# Autodesk Inventor assembly: testRoboRescue_Chassis_Frame
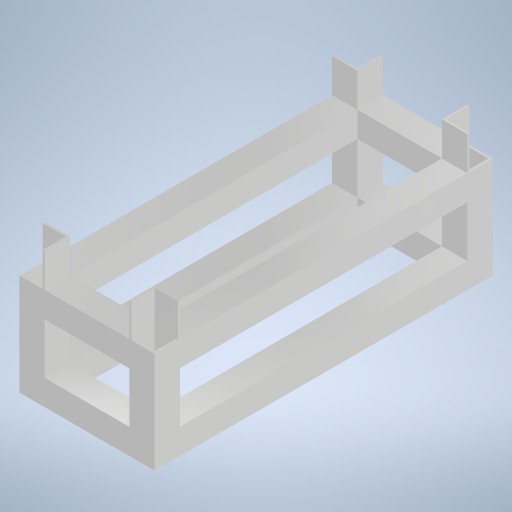
[picture p0: Inventor's stored thumbnail of the model, 512x512]
Saved by Autodesk Inventor 2023 (Build 270158000, 158)
## iProperties
Created: 2022-03-14
Part Number: testRoboRescue_Chassis_Frame
Document SubType Name: Assembly
Designer: Nebil Oumer
Mass: 3473.24 g
Surface Area: 8222.56 cm^2
Volume: 1286.38 cm^3
Author: Nebil Oumer
## Documents named in this file (5)
- C:\Users\seene\Desktop\Stony Brook\SBRT\RoboRescue\Chassis\Frame\testRoboRescue_Chassis_Frame.iam
- RoboRescue_Chassis_Frame.iam
- C:\Users\seene\Desktop\Stony Brook\SBRT\RoboRescue\Chassis\Frame\testRoboRescue_Chassis_Frame_heightBar.ipt
- C:\Users\seene\Desktop\Stony Brook\SBRT\RoboRescue\Chassis\Frame\testRoboRescue_Chassis_Frame_widthBar.ipt
- C:\Users\seene\Desktop\Stony Brook\SBRT\RoboRescue\Chassis\Frame\testRoboRescue_Chassis_Frame_lengthBar.ipt
## Components (12 placed, 3 different names)
1. testRoboRescue_Chassis_Frame_heightBar:1 — Mate:3, Flush:5, Flush:6, Flush:9, Flush:15, Mate:10, Flush:16, Mate:11, Mate:13, Mate:15, Flush:24
2. testRoboRescue_Chassis_Frame_heightBar:2 — Flush:1, Mate:1, Flush:2, Flush:3, Flush:4, Mate:2, Flush:21, Mate:14, Flush:22, Flush:23
3. testRoboRescue_Chassis_Frame_heightBar:3 — Mate:4, Flush:7, Flush:12, Mate:9, Flush:19
4. testRoboRescue_Chassis_Frame_heightBar:4 — Mate:5, Mate:6, Mate:7, Flush:11, Flush:13, Mate:8, Flush:14, Mate:12, Flush:20
5. testRoboRescue_Chassis_Frame_widthBar:1 — Mate:14, Flush:22, Flush:23
6. testRoboRescue_Chassis_Frame_widthBar:2 — Mate:13, Mate:15, Flush:24, Flush:25
7. testRoboRescue_Chassis_Frame_widthBar:3 — Flush:1, Flush:4, Mate:2, Mate:4, Flush:8, Flush:21
8. testRoboRescue_Chassis_Frame_widthBar:4 — Mate:5, Flush:9, Mate:6, Flush:17, Mate:11, Flush:18, Flush:20, Flush:25
9. testRoboRescue_Chassis_Frame_lengthBar:1 — Flush:7, Mate:7, Flush:18, Mate:12, Flush:19
10. testRoboRescue_Chassis_Frame_lengthBar:2 — Flush:15, Mate:10, Flush:16
11. testRoboRescue_Chassis_Frame_lengthBar:3 — Flush:11, Flush:12, Flush:13, Mate:8, Flush:14, Mate:9
12. testRoboRescue_Chassis_Frame_lengthBar:4 — Mate:1, Flush:2, Flush:3, Mate:3, Flush:5, Flush:6, Flush:8, Flush:17
## Relationships (39: Flush 24, Mate 15)
- Flush:1: testRoboRescue_Chassis_Frame_heightBar:2 ↔ testRoboRescue_Chassis_Frame_widthBar:3
- Mate:1: testRoboRescue_Chassis_Frame_heightBar:2 ↔ testRoboRescue_Chassis_Frame_lengthBar:4
- Flush:2: testRoboRescue_Chassis_Frame_heightBar:2 ↔ testRoboRescue_Chassis_Frame_lengthBar:4
- Flush:3: testRoboRescue_Chassis_Frame_heightBar:2 ↔ testRoboRescue_Chassis_Frame_lengthBar:4
- Flush:4: testRoboRescue_Chassis_Frame_heightBar:2 ↔ testRoboRescue_Chassis_Frame_widthBar:3
- Mate:2: testRoboRescue_Chassis_Frame_heightBar:2 ↔ testRoboRescue_Chassis_Frame_widthBar:3
- Mate:3: testRoboRescue_Chassis_Frame_heightBar:1 ↔ testRoboRescue_Chassis_Frame_lengthBar:4
- Flush:5: testRoboRescue_Chassis_Frame_heightBar:1 ↔ testRoboRescue_Chassis_Frame_lengthBar:4
- Flush:6: testRoboRescue_Chassis_Frame_heightBar:1 ↔ testRoboRescue_Chassis_Frame_lengthBar:4
- Mate:4: testRoboRescue_Chassis_Frame_heightBar:3 ↔ testRoboRescue_Chassis_Frame_widthBar:3
- Flush:7: testRoboRescue_Chassis_Frame_heightBar:3 ↔ testRoboRescue_Chassis_Frame_lengthBar:1
- Mate:5: testRoboRescue_Chassis_Frame_heightBar:4 ↔ testRoboRescue_Chassis_Frame_widthBar:4
- Flush:8: testRoboRescue_Chassis_Frame_widthBar:3 ↔ testRoboRescue_Chassis_Frame_lengthBar:4
- Flush:9: testRoboRescue_Chassis_Frame_heightBar:1 ↔ testRoboRescue_Chassis_Frame_widthBar:4
- Mate:6: testRoboRescue_Chassis_Frame_heightBar:4 ↔ testRoboRescue_Chassis_Frame_widthBar:4
- Mate:7: testRoboRescue_Chassis_Frame_heightBar:4 ↔ testRoboRescue_Chassis_Frame_lengthBar:1
- Flush:11: testRoboRescue_Chassis_Frame_heightBar:4 ↔ testRoboRescue_Chassis_Frame_lengthBar:3
- Flush:12: testRoboRescue_Chassis_Frame_heightBar:3 ↔ testRoboRescue_Chassis_Frame_lengthBar:3
- Flush:13: testRoboRescue_Chassis_Frame_heightBar:4 ↔ testRoboRescue_Chassis_Frame_lengthBar:3
- Mate:8: testRoboRescue_Chassis_Frame_heightBar:4 ↔ testRoboRescue_Chassis_Frame_lengthBar:3
- Flush:14: testRoboRescue_Chassis_Frame_heightBar:4 ↔ testRoboRescue_Chassis_Frame_lengthBar:3
- Mate:9: testRoboRescue_Chassis_Frame_heightBar:3 ↔ testRoboRescue_Chassis_Frame_lengthBar:3
- Flush:15: testRoboRescue_Chassis_Frame_heightBar:1 ↔ testRoboRescue_Chassis_Frame_lengthBar:2
- Mate:10: testRoboRescue_Chassis_Frame_heightBar:1 ↔ testRoboRescue_Chassis_Frame_lengthBar:2
- Flush:16: testRoboRescue_Chassis_Frame_heightBar:1 ↔ testRoboRescue_Chassis_Frame_lengthBar:2
- Flush:17: testRoboRescue_Chassis_Frame_widthBar:4 ↔ testRoboRescue_Chassis_Frame_lengthBar:4
- Mate:11: testRoboRescue_Chassis_Frame_heightBar:1 ↔ testRoboRescue_Chassis_Frame_widthBar:4
- Flush:18: testRoboRescue_Chassis_Frame_widthBar:4 ↔ testRoboRescue_Chassis_Frame_lengthBar:1
- Mate:12: testRoboRescue_Chassis_Frame_heightBar:4 ↔ testRoboRescue_Chassis_Frame_lengthBar:1
- Flush:19: testRoboRescue_Chassis_Frame_heightBar:3 ↔ testRoboRescue_Chassis_Frame_lengthBar:1
- Flush:20: testRoboRescue_Chassis_Frame_heightBar:4 ↔ testRoboRescue_Chassis_Frame_widthBar:4
- Mate:13: testRoboRescue_Chassis_Frame_heightBar:1 ↔ testRoboRescue_Chassis_Frame_widthBar:2
- Flush:21: testRoboRescue_Chassis_Frame_heightBar:2 ↔ testRoboRescue_Chassis_Frame_widthBar:3
- Mate:14: testRoboRescue_Chassis_Frame_heightBar:2 ↔ testRoboRescue_Chassis_Frame_widthBar:1
- Flush:22: testRoboRescue_Chassis_Frame_heightBar:2 ↔ testRoboRescue_Chassis_Frame_widthBar:1
- Flush:23: testRoboRescue_Chassis_Frame_heightBar:2 ↔ testRoboRescue_Chassis_Frame_widthBar:1
- Mate:15: testRoboRescue_Chassis_Frame_heightBar:1 ↔ testRoboRescue_Chassis_Frame_widthBar:2
- Flush:24: testRoboRescue_Chassis_Frame_heightBar:1 ↔ testRoboRescue_Chassis_Frame_widthBar:2
- Flush:25: testRoboRescue_Chassis_Frame_widthBar:2 ↔ testRoboRescue_Chassis_Frame_widthBar:4
